# Autodesk Inventor assembly: pasekzkolami
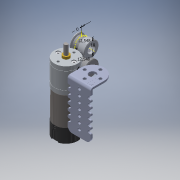
[picture p0: Inventor's stored thumbnail of the model, 180x180]
Saved by Autodesk Inventor 2019 (Build 230136000, 136)
## iProperties
Created: 2020-05-17
Part Number: pasekzkolami
Document SubType Name: Assembly
Designer: estee
Author: estee
## Documents named in this file (8)
- C:\Users\estee\OneDrive\Pulpit\estere\1\MUM\projejt\pasekzkolami.iam
- C:\Users\estee\OneDrive\Pulpit\estere\1\MUM\projejt\przekladnia.ipt
- C:\Users\estee\OneDrive\Pulpit\estere\1\MUM\projejt\zab.ipt
- C:\Users\estee\OneDrive\Pulpit\estere\1\MUM\projejt\pasek.ipt
- C:\Users\estee\OneDrive\Pulpit\estere\1\MUM\projejt\kolooooo.ipt
- C:\Users\estee\OneDrive\Pulpit\estere\1\MUM\projejt\kolo2\GT2_20T-sh8.ipt
- C:\Users\estee\OneDrive\Pulpit\estere\1\MUM\projejt\silnik25d-metal-gearmotor-378-499-encoder.ipt
- C:\Users\estee\OneDrive\Pulpit\estere\1\MUM\projejt\trzymakpololu-25d-mm-metal-gearmotor-bracket.ipt
## Components (44 placed, 7 different names)
1. przekladnia:1 — Flush:1, Flush:2, Flush:3, Mate:1, Angle:1, Mate:2, Angle:2, Mate:3, Mate:4, Mate:5, Mate:7, Mate:9
2. pasek:1 — Mate:3, Mate:4, Mate:5
3. kolooooo:1 — Mate:6, Mate:7, Rotation:1
4. GT2_20T-sh8:1 — Mate:8, Mate:9, Rotation:1
5. silnik25d-metal-gearmotor-378-499-encoder:1
6. trzymakpololu-25d-mm-metal-gearmotor-bracket:1
7. zab:1 — Mate:1, Flush:4, Angle:1
8. zab:2
9. zab:3
10. zab:4
11. zab:5
12. zab:6
13. zab:7
14. zab:8
15. zab:9
16. zab:10
17. zab:11
18. zab:12
19. zab:13
20. zab:14
21. zab:15
22. zab:16
23. zab:17
24. zab:18
25. zab:19
26. zab:20
27. zab:21
28. zab:22
29. zab:23
30. zab:24
31. zab:25
32. zab:26
33. zab:27
34. zab:28
35. zab:29
36. zab:30
37. zab:31
38. zab:32
39. zab:33
40. zab:34
41. zab:35
42. zab:36
43. zab:37
44. zab:38
## Component patterns: (38 elements, first: zab:1)
## Relationships (16: Mate 9, Flush 4, Angle 2, RelateRotation 1)
- Flush:1: przekladnia:1
- Flush:2: przekladnia:1
- Flush:3: przekladnia:1
- Mate:1: przekladnia:1 ↔ zab:1
- Flush:4 (-3 mm): zab:1
- Angle:1 (0 deg): przekladnia:1 ↔ zab:1
- Mate:2: przekladnia:1
- Angle:2 (0 deg): przekladnia:1
- Mate:3: przekladnia:1 ↔ pasek:1
- Mate:4: przekladnia:1 ↔ pasek:1
- Mate:5 (3 mm): przekladnia:1 ↔ pasek:1
- Mate:6: kolooooo:1
- Mate:7 (10.95 mm): przekladnia:1 ↔ kolooooo:1
- Mate:8: GT2_20T-sh8:1
- Mate:9 (10.95 mm): przekladnia:1 ↔ GT2_20T-sh8:1
- Rotation:1 [RelateRotation] (1 ul): kolooooo:1 ↔ GT2_20T-sh8:1
